# Autodesk Inventor assembly: FarmBot
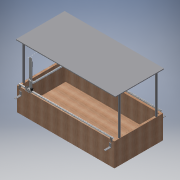
[picture p0: Inventor's stored thumbnail of the model, 180x180]
Saved by Autodesk Inventor 2017 (Build 210142000, 142)
## iProperties
Created: 2016-12-12
Part Number: FarmBot
Document SubType Name: Assembly
Designer: umr
Author: umr
## Documents named in this file (7)
- D:\SeniorProject\Models2\FarmBot.iam
- D:\SeniorProject\Models2\BedAssembly\BedAseembly.iam
- D:\SeniorProject\Models2\Head\HeadSlider.iam
- D:\SeniorProject\Models2\Gantry\GantryDown.iam
- D:\SeniorProject\Models2\Gantry\GantryUp.iam
- D:\SeniorProject\Models2\Case\Case.iam
- D:\SeniorProject\Models2\LED Structure\LED Structure Assembly.iam
## Components (6 placed, 6 different names)
1. BedAseembly:2 [sub-assembly] — Mate:9, Tangent:2, Mate:10, Mate:11, Mate:12, Mate:13, Flush:2, Mate:14, Mate:15, Mate:16
2. HeadSlider:1 [sub-assembly] — Mate:6, Mate:7, Flush:1
3. GantryDown:1 [sub-assembly] — Mate:3, Mate:5, Mate:9, Tangent:2, Flush:2, Flush:3
4. GantryUp:1 [sub-assembly] — Mate:3, Mate:5, Mate:6, Mate:7, Flush:1, Flush:3
5. Case:1 [sub-assembly] — Mate:10, Mate:11, Mate:12, Mate:13
6. LED Structure Assembly:1 [sub-assembly] — Mate:14, Mate:15, Mate:16
## Relationships (16: Mate 12, Flush 3, Tangent 1)
- Mate:3: GantryDown:1 ↔ GantryUp:1
- Mate:5: GantryDown:1 ↔ GantryUp:1
- Mate:6: HeadSlider:1 ↔ GantryUp:1
- Mate:7: HeadSlider:1 ↔ GantryUp:1
- Mate:9: BedAseembly:2 ↔ GantryDown:1
- Tangent:2: BedAseembly:2 ↔ GantryDown:1
- Mate:10: BedAseembly:2 ↔ Case:1
- Mate:11: BedAseembly:2 ↔ Case:1
- Mate:12: BedAseembly:2 ↔ Case:1
- Mate:13: BedAseembly:2 ↔ Case:1
- Flush:1 (50 mm): HeadSlider:1 ↔ GantryUp:1
- Flush:2 (200 mm): BedAseembly:2 ↔ GantryDown:1
- Flush:3 (-200 mm): GantryDown:1 ↔ GantryUp:1
- Mate:14: BedAseembly:2 ↔ LED Structure Assembly:1
- Mate:15: BedAseembly:2 ↔ LED Structure Assembly:1
- Mate:16: BedAseembly:2 ↔ LED Structure Assembly:1
